# Autodesk Inventor assembly: gpsDoor
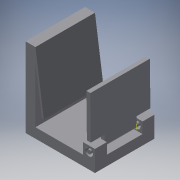
[picture p0: Inventor's stored thumbnail of the model, 180x180]
Saved by Autodesk Inventor 2016 (Build 200138000, 138)
## iProperties
Created: 2016-10-13
Part Number: gpsDoor
Document SubType Name: Assembly
Designer: lachesis
Author: lachesis
## Documents named in this file (3)
- C:\Users\lachesis\git\Swarmie-Build\Swarmie-Assembly\Test_Parts\gpsDoor.iam
- C:\Users\lachesis\git\Swarmie-Build\Swarmie-Assembly\Test_Parts\gpsFrame.ipt
- C:\Users\lachesis\git\Swarmie-Build\Swarmie-Assembly\Test_Parts\gpsDoor.ipt
## Components (2 placed, 2 different names)
1. gpsFrame:1 — Rotational:1
2. gpsDoor:1 — Rotational:1
## Relationships (1: RevoluteJoint 1)
- Rotational:1 [RevoluteJoint]: gpsFrame:1 ↔ gpsDoor:1
